# Autodesk Inventor assembly: 격투로봇
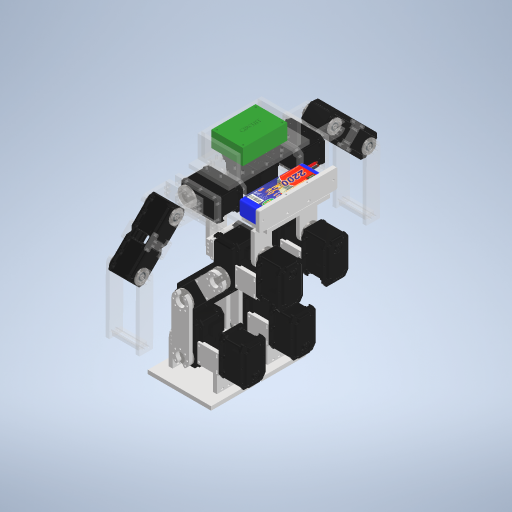
[picture p0: Inventor's stored thumbnail of the model, 512x512]
Saved by Autodesk Inventor 2024.3 (Build 283343000, 343)
## iProperties
Created: 2024-09-16
Part Number: 격투로봇
Document SubType Name: Assembly
Designer: USER
Author: USER
## Documents named in this file (7)
- C:\Users\USER\Desktop\로빛 예비인턴\(git)19기 이원준 격투로봇 설계파일\격투로봇.iam
- C:\Users\USER\Desktop\로빛 예비인턴\(git)19기 이원준 격투로봇 설계파일\Lower_body\고관절\high_joint.iam
- C:\Users\USER\Desktop\로빛 예비인턴\(git)19기 이원준 격투로봇 설계파일\upper_body\팔\left_arm.iam
- C:\Users\USER\Desktop\로빛 예비인턴\(git)19기 이원준 격투로봇 설계파일\Lower_body\다리\left_leg.iam
- C:\Users\USER\Desktop\로빛 예비인턴\(git)19기 이원준 격투로봇 설계파일\upper_body\팔\right_arm.iam
- C:\Users\USER\Desktop\로빛 예비인턴\(git)19기 이원준 격투로봇 설계파일\Lower_body\다리\right_leg.iam
- C:\Users\USER\Desktop\로빛 예비인턴\(git)19기 이원준 격투로봇 설계파일\upper_body\몸체\body.iam
## Components (6 placed, 6 different names)
1. high_joint:1 [sub-assembly] — 각도:3, 각도:6, 삽입:1, 각도:7, 각도:8, 삽입:2
2. left_arm:1 [sub-assembly] — 각도:2, 각도:3, 각도:5, 삽입:3
3. left_leg:1 [sub-assembly] — 플러쉬:2, 플러쉬:3, 각도:7, 각도:8
4. right_arm:1 [sub-assembly] — 각도:1, 각도:2, 각도:4, 각도:5, 삽입:4
5. right_leg:1 [sub-assembly] — 플러쉬:2, 플러쉬:3, 삽입:2
6. body:1 [sub-assembly] — 메이트:1, 플러쉬:1, 각도:6, 삽입:1, 삽입:3, 삽입:4
## Relationships (16: Angle 8, Insert 4, Flush 3, Mate 1)
- 메이트:1 [Mate]: body:1
- 플러쉬:1 [Flush]: body:1
- 각도:1 [Angle] (0 deg): right_arm:1
- 각도:2 [Angle] (0 deg): left_arm:1 ↔ right_arm:1
- 각도:3 [Angle] (0 deg): high_joint:1 ↔ left_arm:1
- 각도:4 [Angle] (0 deg): right_arm:1
- 각도:5 [Angle] (0 deg): left_arm:1 ↔ right_arm:1
- 각도:6 [Angle] (0 deg): high_joint:1 ↔ body:1
- 삽입:1 [Insert]: high_joint:1 ↔ body:1
- 플러쉬:2 [Flush]: left_leg:1 ↔ right_leg:1
- 플러쉬:3 [Flush]: left_leg:1 ↔ right_leg:1
- 각도:7 [Angle] (0 deg): high_joint:1 ↔ left_leg:1
- 각도:8 [Angle] (0 deg): high_joint:1 ↔ left_leg:1
- 삽입:2 [Insert]: high_joint:1 ↔ right_leg:1
- 삽입:3 [Insert]: left_arm:1 ↔ body:1
- 삽입:4 [Insert]: right_arm:1 ↔ body:1
